# Autodesk Inventor assembly: Robot mrk3
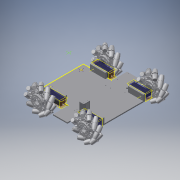
[picture p0: Inventor's stored thumbnail of the model, 180x180]
Saved by Autodesk Inventor 2019 (Build 230136000, 136)
## iProperties
Created: 2017-12-06
Part Number: Robot mrk3
Document SubType Name: Assembly
Designer: User
Author: User
## Documents named in this file (10)
- C:\Robotics\CAD\2018-19_CAD\Robot mrk3.iam
- C:\Robotics\CAD\2017-18_CAD\Prototypes\Gen2PlatePart.ipt
- C:\Robotics\CAD\2017-18_CAD\Prototypes\MecanumWheelFullForVexmotor.iam
- C:\Robotics\CAD\COTSParts\Rev\REV-41-1300HexMotor.ipt
- C:\Robotics\CAD\2017-18_CAD\Prototypes\PossibleTopPlate.ipt
- C:\Robotics\CAD\2017-18_CAD\Prototypes\MotorHolderA.ipt
- C:\Robotics\CAD\2017-18_CAD\Prototypes\MotorHolderB.ipt
- C:\Robotics\CAD\2017-18_CAD\Prototypes\TopPlateRightConnector.ipt
- C:\Robotics\CAD\2017-18_CAD\WheelIntakeBrace.ipt
- C:\Robotics\CAD\2017-18_CAD\Glyph6x6x6.ipt
## Components (18 placed, 9 different names)
1. Gen2PlatePart:1 — Mate:12, Mate:14, Mate:19, Flush:18, Flush:19, Insert:1, Insert:2, Insert:9, Flush:30, Insert:13, Insert:14, Insert:21, Insert:22
2. MecanumWheelFullForVexmotor:1 [sub-assembly] — Insert:24, Rotation:2, Rotation:3
3. MecanumWheelFullForVexmotor:2 [sub-assembly] — Insert:11, Rotation:1
4. MecanumWheelFullForVexmotor:3 [sub-assembly] — Insert:23, Rotation:1, Rotation:3
5. REV-41-1300HexMotor:2 — Mate:12, Mate:24, Insert:23
6. REV-41-1300HexMotor:3 — Mate:14, Mate:20, Mate:21, Insert:24
7. REV-41-1300HexMotor:4 — Insert:11, Insert:20, Angle:1
8. PossibleTopPlate:1 — Mate:19, Flush:18, Flush:19, Mate:38
9. MotorHolderA:1 — Mate:24, Insert:21, Insert:22
10. MotorHolderA:2 — Insert:9, Flush:30, Insert:25, Angle:2
11. MotorHolderB:1 — Mate:20, Mate:21, Mate:39, Flush:21
12. MotorHolderB:2 — Insert:13, Insert:14, Insert:20, Angle:1
13. TopPlateRightConnector:1 — Mate:38, Mate:39, Flush:21
14. WheelIntakeBrace:1 — Insert:1, Insert:2
15. REV-41-1300HexMotor:5 — Insert:25, Angle:2, Insert:26
16. MecanumWheelFullForVexmotor:4 [sub-assembly] — Insert:26, Rotation:2
17. Glyph6x6x6:1
18. Glyph6x6x6:2
## Relationships (30: Insert 13, Mate 8, Flush 4, RelateRotation 3, Angle 2)
- Mate:12: Gen2PlatePart:1 ↔ REV-41-1300HexMotor:2
- Mate:14: Gen2PlatePart:1 ↔ REV-41-1300HexMotor:3
- Mate:19 (254 mm): Gen2PlatePart:1 ↔ PossibleTopPlate:1
- Flush:18: Gen2PlatePart:1 ↔ PossibleTopPlate:1
- Flush:19: Gen2PlatePart:1 ↔ PossibleTopPlate:1
- Mate:20: REV-41-1300HexMotor:3 ↔ MotorHolderB:1
- Mate:21: REV-41-1300HexMotor:3 ↔ MotorHolderB:1
- Mate:24: REV-41-1300HexMotor:2 ↔ MotorHolderA:1
- Mate:38: PossibleTopPlate:1 ↔ TopPlateRightConnector:1
- Mate:39: MotorHolderB:1 ↔ TopPlateRightConnector:1
- Flush:21: MotorHolderB:1 ↔ TopPlateRightConnector:1
- Insert:1: Gen2PlatePart:1 ↔ WheelIntakeBrace:1
- Insert:2: Gen2PlatePart:1 ↔ WheelIntakeBrace:1
- Insert:9: Gen2PlatePart:1 ↔ MotorHolderA:2
- Flush:30: Gen2PlatePart:1 ↔ MotorHolderA:2
- Insert:11: MecanumWheelFullForVexmotor:2 ↔ REV-41-1300HexMotor:4
- Insert:13: Gen2PlatePart:1 ↔ MotorHolderB:2
- Insert:14: Gen2PlatePart:1 ↔ MotorHolderB:2
- Insert:20: REV-41-1300HexMotor:4 ↔ MotorHolderB:2
- Angle:1 (180 deg): REV-41-1300HexMotor:4 ↔ MotorHolderB:2
- Insert:21: Gen2PlatePart:1 ↔ MotorHolderA:1
- Insert:22: Gen2PlatePart:1 ↔ MotorHolderA:1
- Insert:23: MecanumWheelFullForVexmotor:3 ↔ REV-41-1300HexMotor:2
- Insert:24: MecanumWheelFullForVexmotor:1 ↔ REV-41-1300HexMotor:3
- Insert:25: MotorHolderA:2 ↔ REV-41-1300HexMotor:5
- Angle:2 (0 deg): MotorHolderA:2 ↔ REV-41-1300HexMotor:5
- Insert:26: REV-41-1300HexMotor:5 ↔ MecanumWheelFullForVexmotor:4
- Rotation:1 [RelateRotation] (1 ul): MecanumWheelFullForVexmotor:2 ↔ MecanumWheelFullForVexmotor:3
- Rotation:2 [RelateRotation] (1 ul): MecanumWheelFullForVexmotor:1 ↔ MecanumWheelFullForVexmotor:4
- Rotation:3 [RelateRotation] (1 ul): MecanumWheelFullForVexmotor:1 ↔ MecanumWheelFullForVexmotor:3
